# Autodesk Inventor assembly: IntakeSide
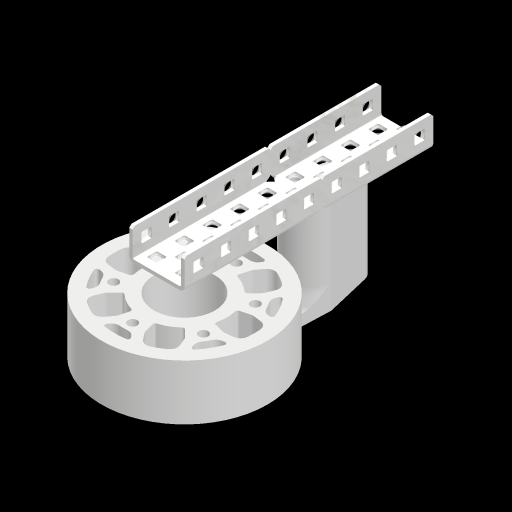
[picture p0: Inventor's stored thumbnail of the model, 512x512]
Saved by Autodesk Inventor 2024.1 (Build 281209000, 209)
## iProperties
Created: 2025-05-12
Part Number: IntakeSide
Document SubType Name: Assembly
Designer: Teddy
Author: Teddy
## Documents named in this file (5)
- C:\Users\Teddy\OneDrive\Desktop\VEX-CAD-Inventor-1.4.0\pushBack\IntakeSide.iam
- C:\Users\Teddy\OneDrive\Desktop\VEX-CAD-Inventor-1.4.0\Motion\Wheels\Flex Wheels\3.000 Flex Wheel\3.000 30A 1.000.ipt
- C:\Users\Teddy\OneDrive\Desktop\VEX-CAD-Inventor-1.4.0\Motion\Wheels\Flex Wheels\3.000 Flex Wheel.ipt
- C:\Users\Teddy\OneDrive\Desktop\VEX-CAD-Inventor-1.4.0\Structure\C Channel\Aluminum 1x2x1\Alu C 1x2x1x9.ipt
- C:\Users\Teddy\OneDrive\Desktop\VEX-CAD-Inventor-1.4.0\pushBack\IntakeRotator.ipt
## Components (3 placed, 3 different names)
1. 3.000 30A 1.000:1 — Insert:1, Flush:1, Flush:2
2. Alu C 1x2x1x9:1 — Insert:1
3. IntakeRotator:1 — Flush:1, Flush:2
## Relationships (3: Flush 2, Insert 1)
- Insert:1 (12.7 mm): 3.000 30A 1.000:1 ↔ Alu C 1x2x1x9:1
- Flush:1: 3.000 30A 1.000:1 ↔ IntakeRotator:1
- Flush:2: 3.000 30A 1.000:1 ↔ IntakeRotator:1
